# Autodesk Inventor assembly: Assembly2
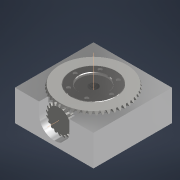
[picture p0: Inventor's stored thumbnail of the model, 180x180]
Saved by Autodesk Inventor 2022 (Build 260153000, 153)
## iProperties
Part Number: Assembly2
Document SubType Name: Assembly
Designer: Andres
Author: Andres
## Documents named in this file (6)
- D:\Documentos\15.PUCP_2021-2\[PDM] Proyecto de Diseño Mecatrónico\ProyectoGIT\ProyectoRobotPallet\SistemaDeElevación\version2\Assembly2.iam
- D:\Documentos\15.PUCP_2021-2\[PDM] Proyecto de Diseño Mecatrónico\ProyectoGIT\ProyectoRobotPallet\SistemaDeElevación\version2\Soporte.ipt
- D:\Documentos\15.PUCP_2021-2\[PDM] Proyecto de Diseño Mecatrónico\ProyectoGIT\ProyectoRobotPallet\SistemaDeElevación\version2\Tuerca3.ipt
- D:\Documentos\15.PUCP_2021-2\[PDM] Proyecto de Diseño Mecatrónico\ProyectoGIT\ProyectoRobotPallet\SistemaDeElevación\AIS2021\SKF_7205 BE-2RZP.iam
- D:\Documentos\15.PUCP_2021-2\[PDM] Proyecto de Diseño Mecatrónico\ProyectoGIT\ProyectoRobotPallet\SistemaDeElevación\version2\Assembly2\Design Accelerator\Bevel Gears3.iam
- D:\Documentos\15.PUCP_2021-2\[PDM] Proyecto de Diseño Mecatrónico\ProyectoGIT\ProyectoRobotPallet\SistemaDeElevación\version2\SeguroRodamientos.ipt
## Components (6 placed, 5 different names)
1. Soporte:1 — Flush:1, Mate:3, Mate:4, Mate:6, Flush:2
2. Tuerca3:1 — Flush:1, Mate:5, Angle:1
3. SKF_7205 BE-2RZP:1 [sub-assembly] — Mate:1, Mate:2, Mate:3, Mate:4
4. SKF_7205 BE-2RZP:2 [sub-assembly] — Mate:1, Mate:2
5. Bevel Gears:1 [sub-assembly] — Mate:5, Angle:1, Mate:6
6. SeguroRodamientos:1 — Flush:2
## Relationships (9: Mate 6, Flush 2, Angle 1)
- Flush:1: Soporte:1 ↔ Tuerca3:1
- Mate:1: SKF_7205 BE-2RZP:1 ↔ SKF_7205 BE-2RZP:2
- Mate:2: SKF_7205 BE-2RZP:1 ↔ SKF_7205 BE-2RZP:2
- Mate:3: Soporte:1 ↔ SKF_7205 BE-2RZP:1
- Mate:4: Soporte:1 ↔ SKF_7205 BE-2RZP:1
- Mate:5: Tuerca3:1 ↔ Bevel Gears:1
- Angle:1 (0 deg): Tuerca3:1 ↔ Bevel Gears:1
- Mate:6: Soporte:1 ↔ Bevel Gears:1
- Flush:2: Soporte:1 ↔ SeguroRodamientos:1
